# Autodesk Inventor assembly: сборка_v1
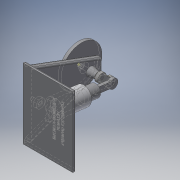
[picture p0: Inventor's stored thumbnail of the model, 180x180]
Saved by Autodesk Inventor 2017.3 (Build 213256000, 256)
## iProperties
Part Number: сборка_v1
Material: Типовые
Document SubType Name: Assembly
Designer: Alexnav
Author: Alexnav
## Documents named in this file (8)
- E:\Study\4sem\appmech\homework\1\src\5\сборка\сборка_v2.iam
- E:\Study\4sem\appmech\homework\1\src\5\кривошип\кривошип_v1.ipt
- E:\Study\4sem\appmech\homework\1\src\5\маховик\маховик_v1.ipt
- E:\Study\4sem\appmech\homework\1\src\5\вал\вал_v1.ipt
- E:\Study\4sem\appmech\homework\1\src\5\вал\вал2_v1.ipt
- E:\Study\4sem\appmech\homework\1\src\5\камень\стакан_v2.ipt
- E:\Study\4sem\appmech\homework\1\src\5\cтойка\стойка_v2.ipt
- E:\Study\4sem\appmech\homework\1\src\5\кулиса\поршень_v2.ipt
## Components (7 placed, 7 different names)
1. кривошип_v1:1 — Жесткий:2, Жесткий:3
2. маховик_v1:1 — Жесткий:1
3. вал_v1:1 — Жесткий:1, Жесткий:2, Цилиндрический:4
4. вал2_v1:1 — Жесткий:3, Цилиндрический:5
5. стакан_v2:1 — С поворотом:1, Цилиндрический:6
6. стойка_v2:1 — Цилиндрический:4, С поворотом:1, Совмещение:1, Совмещение:2, Совмещение:3
7. поршень_v2:1 — Цилиндрический:5, Цилиндрический:6
## Relationships (10: WeldJoint 3, CylindricalJoint 3, Mate 3, RevoluteJoint 1)
- Жесткий:1 [WeldJoint]: маховик_v1:1 ↔ вал_v1:1
- Жесткий:2 [WeldJoint] (-10 mm): кривошип_v1:1 ↔ вал_v1:1
- Жесткий:3 [WeldJoint] (10 mm): кривошип_v1:1 ↔ вал2_v1:1
- Цилиндрический:4 [CylindricalJoint]: вал_v1:1 ↔ стойка_v2:1
- С поворотом:1 [RevoluteJoint] (30 mm): стакан_v2:1 ↔ стойка_v2:1
- Совмещение:1 [Mate]: стойка_v2:1
- Совмещение:2 [Mate]: стойка_v2:1
- Совмещение:3 [Mate]: стойка_v2:1
- Цилиндрический:5 [CylindricalJoint]: вал2_v1:1 ↔ поршень_v2:1
- Цилиндрический:6 [CylindricalJoint]: стакан_v2:1 ↔ поршень_v2:1
## Named parameters: Временная_шкала_моделирования = 0
